# Autodesk Inventor assembly: nema17-soporte
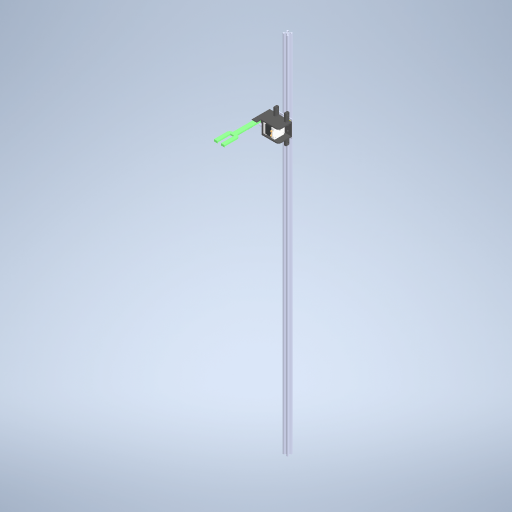
[picture p0: Inventor's stored thumbnail of the model, 512x512]
Saved by Autodesk Inventor 2024.3 (Build 283343000, 343)
## iProperties
Created: 2024-11-02
Part Number: nema17-soporte
Description: FreeCAD Model
Document SubType Name: Assembly
Designer: cjoao
Authority: Unknown
Sending System: FreeCAD
Preprocessor: Open CASCADE STEP processor 7.6
Title: Open CASCADE Shape Model
## Documents named in this file (7)
- C:\Users\cjoao\OneDrive\Desktop\TESIS\actuadorZ\nema17-soporte.iam
- C:\Users\cjoao\OneDrive\Desktop\TESIS\actuadorZ\Body.ipt
- C:\Users\cjoao\OneDrive\Desktop\TESIS\V-Slot 20-20-2016_placa plana.ipt
- C:\Users\cjoao\OneDrive\Desktop\TESIS\Nima 17 40x42x5mm.ipt
- C:\Users\cjoao\OneDrive\Desktop\TESIS\actuadorZ\piñon.ipt
- C:\Users\cjoao\OneDrive\Desktop\TESIS\actuadorZ\cremallera 150.ipt
- C:\Users\cjoao\OneDrive\Desktop\TESIS\soportes eje y poleas\Ensamblaje2.iam
## Components (6 placed, 6 different names)
1. Body — Coincidencia:1, Coincidencia:3, Coincidencia:4, Coincidencia:7, Coincidencia:8, Coincidencia:10, Coincidencia:11, Coincidencia:12
2. V-Slot 20-20-2016_placa plana:1 — Coincidencia:1, Coincidencia:9, Nivelación:2, Coincidencia:10, Coincidencia:11, Coincidencia:12
3. Nima 17 40x42x5mm:1 — Coincidencia:3, Coincidencia:4, Coincidencia:5, Coincidencia:6
4. piñon:1 — Coincidencia:5, Coincidencia:6
5. cremallera 150:1 — Coincidencia:7, Coincidencia:8
6. Ensamblaje2:1 [sub-assembly] — Coincidencia:9, Nivelación:2
## Relationships (12: Mate 11, Flush 1)
- Coincidencia:1 [Mate]: Body ↔ V-Slot 20-20-2016_placa plana:1
- Coincidencia:3 [Mate]: Body ↔ Nima 17 40x42x5mm:1
- Coincidencia:4 [Mate]: Body ↔ Nima 17 40x42x5mm:1
- Coincidencia:5 [Mate]: Nima 17 40x42x5mm:1 ↔ piñon:1
- Coincidencia:6 [Mate]: Nima 17 40x42x5mm:1 ↔ piñon:1
- Coincidencia:7 [Mate]: Body ↔ cremallera 150:1
- Coincidencia:8 [Mate]: Body ↔ cremallera 150:1
- Coincidencia:9 [Mate]: V-Slot 20-20-2016_placa plana:1 ↔ Ensamblaje2:1
- Nivelación:2 [Flush]: V-Slot 20-20-2016_placa plana:1 ↔ Ensamblaje2:1
- Coincidencia:10 [Mate]: Body ↔ V-Slot 20-20-2016_placa plana:1
- Coincidencia:11 [Mate]: Body ↔ V-Slot 20-20-2016_placa plana:1
- Coincidencia:12 [Mate]: Body ↔ V-Slot 20-20-2016_placa plana:1
